# Autodesk Inventor assembly: 3-finger_gripper
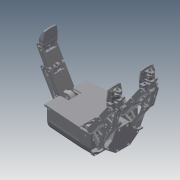
[picture p0: Inventor's stored thumbnail of the model, 180x180]
Saved by Autodesk Inventor 2018 (Build 220112000, 112)
## iProperties
Created: 2019-01-30
Part Number: 3-finger_gripper
Document SubType Name: Assembly
Designer: Tsche
Author: Tsche
## Documents named in this file (26)
- C:\Users\Tsche\Documents\3d-printer\parts\grippers\Three_Finger_Gripper\BetaBots-Robot-Arm-Project-master\BetaBots-Robot-Arm-Project-master\ThreeFingerGripper\inventor\Gripper\cad_files\3-finger_gripper.iam
- C:\Users\Tsche\Documents\3d-printer\parts\grippers\Three_Finger_Gripper\BetaBots-Robot-Arm-Project-master\BetaBots-Robot-Arm-Project-master\ThreeFingerGripper\inventor\Gripper\cad_files\finger_part_a.ipt
- C:\Users\Tsche\Documents\3d-printer\parts\grippers\Three_Finger_Gripper\BetaBots-Robot-Arm-Project-master\BetaBots-Robot-Arm-Project-master\ThreeFingerGripper\inventor\Gripper\cad_files\finger_part_b.ipt
- C:\Users\Tsche\Documents\3d-printer\parts\grippers\Three_Finger_Gripper\BetaBots-Robot-Arm-Project-master\BetaBots-Robot-Arm-Project-master\ThreeFingerGripper\inventor\Gripper\cad_files\finger_part_c.ipt
- C:\Users\Tsche\Documents\3d-printer\parts\grippers\Three_Finger_Gripper\BetaBots-Robot-Arm-Project-master\BetaBots-Robot-Arm-Project-master\ThreeFingerGripper\inventor\Gripper\cad_files\bar_bc.ipt
- C:\Users\Tsche\Documents\3d-printer\parts\grippers\Three_Finger_Gripper\BetaBots-Robot-Arm-Project-master\BetaBots-Robot-Arm-Project-master\ThreeFingerGripper\inventor\Gripper\cad_files\hinge_act_b.ipt
- C:\Users\Tsche\Documents\3d-printer\parts\grippers\Three_Finger_Gripper\BetaBots-Robot-Arm-Project-master\BetaBots-Robot-Arm-Project-master\ThreeFingerGripper\inventor\Gripper\cad_files\bar_act_ab.ipt
- C:\Users\Tsche\Documents\3d-printer\parts\grippers\Three_Finger_Gripper\BetaBots-Robot-Arm-Project-master\BetaBots-Robot-Arm-Project-master\ThreeFingerGripper\inventor\Gripper\cad_files\hinge_guid_b.ipt
- C:\Users\Tsche\Documents\3d-printer\parts\grippers\Three_Finger_Gripper\BetaBots-Robot-Arm-Project-master\BetaBots-Robot-Arm-Project-master\ThreeFingerGripper\inventor\Gripper\cad_files\bar_guid_ab.ipt
- C:\Users\Tsche\Documents\3d-printer\parts\grippers\Three_Finger_Gripper\BetaBots-Robot-Arm-Project-master\BetaBots-Robot-Arm-Project-master\ThreeFingerGripper\inventor\Gripper\cad_files\hinge_guid_a.ipt
- C:\Users\Tsche\Documents\3d-printer\parts\grippers\Three_Finger_Gripper\BetaBots-Robot-Arm-Project-master\BetaBots-Robot-Arm-Project-master\ThreeFingerGripper\inventor\Gripper\cad_files\hinge_guid_c.ipt
- C:\Users\Tsche\Documents\3d-printer\parts\grippers\Three_Finger_Gripper\BetaBots-Robot-Arm-Project-master\BetaBots-Robot-Arm-Project-master\ThreeFingerGripper\inventor\Gripper\cad_files\hinge_act_a2.ipt
- C:\Users\Tsche\Documents\3d-printer\parts\grippers\Three_Finger_Gripper\BetaBots-Robot-Arm-Project-master\BetaBots-Robot-Arm-Project-master\ThreeFingerGripper\inventor\Gripper\cad_files\worm.ipt
- C:\Users\Tsche\Documents\3d-printer\parts\grippers\Three_Finger_Gripper\BetaBots-Robot-Arm-Project-master\BetaBots-Robot-Arm-Project-master\ThreeFingerGripper\inventor\Gripper\cad_files\dc-motor_12V_60U-min.ipt
- C:\Users\Tsche\Documents\3d-printer\parts\grippers\Three_Finger_Gripper\BetaBots-Robot-Arm-Project-master\BetaBots-Robot-Arm-Project-master\ThreeFingerGripper\inventor\Gripper\cad_files\3-finger_gripper_finger_B.iam
- C:\Users\Tsche\Documents\3d-printer\parts\grippers\Three_Finger_Gripper\BetaBots-Robot-Arm-Project-master\BetaBots-Robot-Arm-Project-master\ThreeFingerGripper\inventor\Gripper\cad_files\servo_ES08MA2.ipt
- C:\Users\Tsche\Documents\3d-printer\parts\grippers\Three_Finger_Gripper\BetaBots-Robot-Arm-Project-master\BetaBots-Robot-Arm-Project-master\ThreeFingerGripper\inventor\Gripper\cad_files\tilt-gear_A_servo.ipt
- C:\Users\Tsche\Documents\3d-printer\parts\grippers\Three_Finger_Gripper\BetaBots-Robot-Arm-Project-master\BetaBots-Robot-Arm-Project-master\ThreeFingerGripper\inventor\Gripper\cad_files\tilt-guide.ipt
- C:\Users\Tsche\Documents\3d-printer\parts\grippers\Three_Finger_Gripper\BetaBots-Robot-Arm-Project-master\BetaBots-Robot-Arm-Project-master\ThreeFingerGripper\inventor\Gripper\cad_files\finger-main_A.ipt
- C:\Users\Tsche\Documents\3d-printer\parts\grippers\Three_Finger_Gripper\BetaBots-Robot-Arm-Project-master\BetaBots-Robot-Arm-Project-master\ThreeFingerGripper\inventor\Gripper\cad_files\Design Accelerator\Spur Gears2.iam
- C:\Users\Tsche\Documents\3d-printer\parts\grippers\Three_Finger_Gripper\BetaBots-Robot-Arm-Project-master\BetaBots-Robot-Arm-Project-master\ThreeFingerGripper\inventor\Gripper\cad_files\Design Accelerator\Spur Gears3.iam
- C:\Users\Tsche\Documents\3d-printer\parts\grippers\Three_Finger_Gripper\BetaBots-Robot-Arm-Project-master\BetaBots-Robot-Arm-Project-master\ThreeFingerGripper\inventor\Gripper\cad_files\tilt-axis_mount.ipt
- C:\Users\Tsche\Documents\3d-printer\parts\grippers\Three_Finger_Gripper\BetaBots-Robot-Arm-Project-master\BetaBots-Robot-Arm-Project-master\ThreeFingerGripper\inventor\Gripper\cad_files\3-finger_gripper_finger_C.iam
- C:\Users\Tsche\Documents\3d-printer\parts\grippers\Three_Finger_Gripper\BetaBots-Robot-Arm-Project-master\BetaBots-Robot-Arm-Project-master\ThreeFingerGripper\inventor\Gripper\cad_files\finger-tip_base.ipt
- C:\Users\Tsche\Documents\3d-printer\parts\grippers\Three_Finger_Gripper\BetaBots-Robot-Arm-Project-master\BetaBots-Robot-Arm-Project-master\ThreeFingerGripper\inventor\Gripper\cad_files\hand-palm.ipt
- C:\Users\Tsche\Documents\3d-printer\parts\grippers\Three_Finger_Gripper\BetaBots-Robot-Arm-Project-master\BetaBots-Robot-Arm-Project-master\ThreeFingerGripper\inventor\Gripper\cad_files\Dimensions.xlsx
## Components (26 placed, 23 different names)
1. finger-main_A:1 — Cylindrical:20, Flush:12, Cylindrical:21, Mate:15, Angle:1, Mate:16, Mate:19, Flush:24, Mate:22, Flush:30, Mate:31, Mate:36, Mate:41, Angle:4, Mate:44, Mate:45, Mate:46, Mate:47, Mate:48, Mate:49, Angle:5, Cylindrical:16, Cylindrical:19
2. finger_part_a:1 — Cylindrical:1, Flush:1, Cylindrical:20, Flush:12, Mate:14
3. finger_part_b:1 — Cylindrical:1, Flush:1, Cylindrical:2, Mate:3, Cylindrical:4, Cylindrical:9
4. finger_part_c:1 — Cylindrical:2, Mate:3, Mate:4, Cylindrical:3, Cylindrical:14, Flush:31, Mate:52, Flush:32
5. finger-tip_base:1 — Flush:31, Mate:52, Flush:32
6. bar_bc:1 — Mate:4, Cylindrical:3, Mate:5, Cylindrical:5, Mate:6, Flush:2
7. hinge_act_b:1 — Mate:5, Cylindrical:4, Cylindrical:5, Cylindrical:6
8. bar_act_ab:1 — Mate:6, Cylindrical:6, Mate:13, Cylindrical:18
9. bar_bc:2 — Flush:2, Mate:8, Cylindrical:10, Mate:11, Cylindrical:15
10. hinge_guid_b:1 — Mate:8, Cylindrical:9, Cylindrical:10, Mate:9, Cylindrical:11
11. bar_guid_ab:1 — Mate:9, Cylindrical:11, Flush:11, Cylindrical:17
12. hinge_guid_a:1 — Flush:11, Cylindrical:16, Cylindrical:17
13. hinge_guid_c:1 — Mate:11, Cylindrical:14, Cylindrical:15
14. Worm Gear:1 — Mate:13, Cylindrical:18, Cylindrical:19
15. Worm:2 — Cylindrical:21, Mate:14
16. dc-motor_12V_60U-min:1 — Mate:15, Angle:1, Mate:16
17. servo_ES08MA2:1 — Mate:19, Mate:21, Cylindrical:22, Flush:24, Mate:22, Mate:39
18. tilt-gear_A_servo:1 — Mate:21, Cylindrical:22
19. tilt-guide:1 — Flush:30, Mate:31, Mate:41, Mate:42, Mate:43, Mate:51
20. 3-finger_gripper_finger_B:1 [sub-assembly] — Mate:42, Mate:43, Angle:4, Flush:51
21. 3-finger_gripper_finger_C:1 [sub-assembly] — Flush:51, Mate:51, Angle:5
22. Spur Gears:1 [sub-assembly] — Mate:36, Flush:16
23. Spur Gears:2 [sub-assembly] — Mate:39
24. tilt-axis_mount:1 — Mate:44, Mate:45, Mate:46
25. tilt-axis_mount:2 — Mate:47, Mate:48, Mate:49
26. hand-palm:1 — Mate:53, Mate:54, Flush:33
## Relationships (62: Mate 30, CylindricalJoint 18, Flush 11, Angle 3)
- Cylindrical:1: finger_part_a:1 ↔ finger_part_b:1
- Flush:1: finger_part_a:1 ↔ finger_part_b:1
- Cylindrical:2: finger_part_b:1 ↔ finger_part_c:1
- Mate:3: finger_part_b:1 ↔ finger_part_c:1
- Mate:4: finger_part_c:1 ↔ bar_bc:1
- Cylindrical:3: finger_part_c:1 ↔ bar_bc:1
- Mate:5: bar_bc:1 ↔ hinge_act_b:1
- Cylindrical:4: finger_part_b:1 ↔ hinge_act_b:1
- Cylindrical:5: bar_bc:1 ↔ hinge_act_b:1
- Mate:6: bar_bc:1 ↔ bar_act_ab:1
- Cylindrical:6: hinge_act_b:1 ↔ bar_act_ab:1
- Flush:2 (8 mm): bar_bc:1 ↔ bar_bc:2
- Mate:8: bar_bc:2 ↔ hinge_guid_b:1
- Cylindrical:9: finger_part_b:1 ↔ hinge_guid_b:1
- Cylindrical:10: bar_bc:2 ↔ hinge_guid_b:1
- Mate:9: hinge_guid_b:1 ↔ bar_guid_ab:1
- Cylindrical:11: hinge_guid_b:1 ↔ bar_guid_ab:1
- Flush:11: bar_guid_ab:1 ↔ hinge_guid_a:1
- Mate:11: bar_bc:2 ↔ hinge_guid_c:1
- Cylindrical:14: finger_part_c:1 ↔ hinge_guid_c:1
- Cylindrical:15: bar_bc:2 ↔ hinge_guid_c:1
- Cylindrical:16: finger-main_A:1 ↔ hinge_guid_a:1
- Cylindrical:17: bar_guid_ab:1 ↔ hinge_guid_a:1
- Mate:13: bar_act_ab:1 ↔ Worm Gear:1
- Cylindrical:18: bar_act_ab:1 ↔ Worm Gear:1
- Cylindrical:19: finger-main_A:1 ↔ Worm Gear:1
- Cylindrical:20: finger-main_A:1 ↔ finger_part_a:1
- Flush:12: finger-main_A:1 ↔ finger_part_a:1
- Cylindrical:21: finger-main_A:1 ↔ Worm:2
- Mate:14: finger_part_a:1 ↔ Worm:2
- Mate:15: finger-main_A:1 ↔ dc-motor_12V_60U-min:1
- Angle:1 (0 deg): finger-main_A:1 ↔ dc-motor_12V_60U-min:1
- Mate:16: finger-main_A:1 ↔ dc-motor_12V_60U-min:1
- Mate:19: finger-main_A:1 ↔ servo_ES08MA2:1
- Mate:21 (0.2 mm): servo_ES08MA2:1 ↔ tilt-gear_A_servo:1
- Cylindrical:22: servo_ES08MA2:1 ↔ tilt-gear_A_servo:1
- Flush:24 (-1 mm): finger-main_A:1 ↔ servo_ES08MA2:1
- Mate:22 (-10 mm): finger-main_A:1 ↔ servo_ES08MA2:1
- Flush:30: finger-main_A:1 ↔ tilt-guide:1
- Mate:31 (15 mm): finger-main_A:1 ↔ tilt-guide:1
- Mate:36: finger-main_A:1 ↔ Spur Gears:1
- Flush:16 (25.625 mm): Spur Gears:1
- Mate:39: servo_ES08MA2:1 ↔ Spur Gears:2
- Mate:41: finger-main_A:1 ↔ tilt-guide:1
- Mate:42 (0.15 mm): tilt-guide:1 ↔ 3-finger_gripper_finger_B:1
- Mate:43: tilt-guide:1 ↔ 3-finger_gripper_finger_B:1
- Angle:4 (0 deg): finger-main_A:1 ↔ 3-finger_gripper_finger_B:1
- Mate:44: finger-main_A:1 ↔ tilt-axis_mount:1
- Mate:45: finger-main_A:1 ↔ tilt-axis_mount:1
- Mate:46: finger-main_A:1 ↔ tilt-axis_mount:1
- Mate:47: finger-main_A:1 ↔ tilt-axis_mount:2
- Mate:48: finger-main_A:1 ↔ tilt-axis_mount:2
- Mate:49: finger-main_A:1 ↔ tilt-axis_mount:2
- Flush:51: 3-finger_gripper_finger_B:1 ↔ 3-finger_gripper_finger_C:1
- Mate:51: tilt-guide:1 ↔ 3-finger_gripper_finger_C:1
- Angle:5 (0 deg): finger-main_A:1 ↔ 3-finger_gripper_finger_C:1
- Flush:31: finger_part_c:1 ↔ finger-tip_base:1
- Mate:52: finger_part_c:1 ↔ finger-tip_base:1
- Flush:32: finger_part_c:1 ↔ finger-tip_base:1
- Mate:53 (0.65 mm): hand-palm:1
- Mate:54: hand-palm:1
- Flush:33 (-35 mm): hand-palm:1
## Named parameters: finger_width = 25 mm, finger_thickness = 8 mm, finger_part_A_length = 42.8625 mm, finger_part_B_length = 28.575 mm, finger_link_width = 3.5 mm, finger_link_clearence = 0.075 mm, tol = 0.0375 mm, link_tol = 0.254 mm, bore_press = 2.925 mm, bore_clearance = 3.025 mm, bar_diameter = 6.5 mm, bar_thickness = 4 mm, bar_width = 7 mm, hinge_dist_sym_plane = 4 mm, hinge_thickness = 3 mm, hinge_act_length_c = 7.62 mm, hinge_act_length_bc = 16.66875 mm, hinge_act_length_ab = 11.049 mm, hinge_act_length_a = 21.43125 mm, hinge_guid_length_c = 9.525 mm, hinge_guid_length_bc = 9.525 mm, hinge_guid_length_ab = 17.145 mm, hinge_guid_length_a = 17.145 mm, bar_length_bc = 28.575 mm, bar_act_length_ab = 40.48125 mm, bar_guid_length_ab = 43.275 mm, champfer = 0.3 mm, fillet = 0.4 mm, gear_diameter = 14 mm, dist_finger_BC = 56.5 mm, dist_hinge_points = 51.25 mm, hinge_point = 15 mm
